# Autodesk Inventor assembly: Assembly1
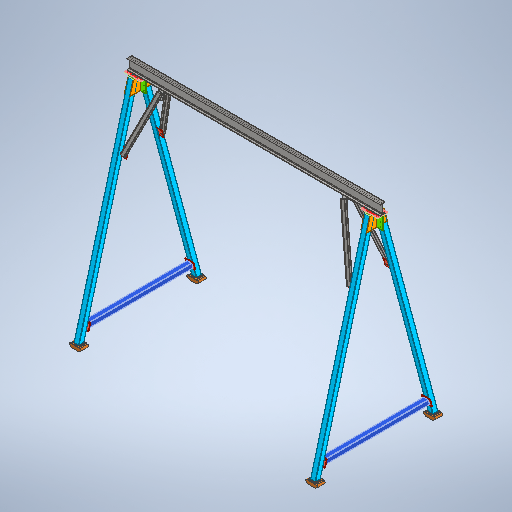
[picture p0: Inventor's stored thumbnail of the model, 512x512]
Saved by Autodesk Inventor 2025 (Build 290162010, 162A)
## iProperties
Created: 2024-06-11
Part Number: Assembly1
Document SubType Name: Assembly
Designer: admin
Author: admin
## Documents named in this file (6)
- C:\Users\pokla\Documents\Inventor\Goat 1\Assembly1.iam
- C:\Users\pokla\Documents\Inventor\Goat 1\WRS 000,000 кран козловой 6х4.ipt
- C:\Users\pokla\Documents\Inventor\Goat 1\Тельфер Таль электрическая.ipt
- C:\Users\pokla\Documents\Inventor\Goat 1\Сrane plate 1.ipt
- C:\Users\pokla\Documents\Inventor\Goat 1\Assembly2 стойка.iam
- C:\Users\pokla\Documents\Inventor\Goat 1\Двутавр 240x36 - 6000.ipt
## Components (7 placed, 7 different names)
1. WRS 000,000 кран козловой 6х4.ipt:1 — Mate:2, Mate:3, Flush:3
2. Тельфер Таль электрическая.ipt:1 — Mate:4
3. Сrane plate 1.ipt:1 — Flush:18
4. Assembly2 стойка.iam:1 [sub-assembly] — Flush:24, Flush:25, Flush:26
5. Двутавр 240x36 - 6000:1 — Mate:7, Mate:8, Flush:28
6. Assembly2 стойка:2 [sub-assembly] — Flush:27, Mate:5, Mate:6, Rigid:3
7. Сrane plate 1:2 — Rigid:3, Mate:8
## Relationships (18: Flush 9, Mate 7, WeldJoint 2)
- Mate:2: WRS 000,000 кран козловой 6х4.ipt:1
- Mate:3: WRS 000,000 кран козловой 6х4.ipt:1
- Flush:3: WRS 000,000 кран козловой 6х4.ipt:1
- Mate:4: Тельфер Таль электрическая.ipt:1
- [Flush]: Assembly2 стойка.iam:1
- Flush:18: Сrane plate 1.ipt:1
- [Flush]: Assembly2 стойка.iam:1
- [WeldJoint]: Сrane plate 1.ipt:1 ↔ Assembly2 стойка.iam:1
- Flush:24: Assembly2 стойка.iam:1
- Flush:25: Assembly2 стойка.iam:1
- Flush:26 (-2800 mm): Assembly2 стойка.iam:1
- Flush:27: Assembly2 стойка:2
- Mate:5: Assembly2 стойка:2
- Mate:6 (-2800 mm): Assembly2 стойка:2
- Rigid:3 [WeldJoint]: Assembly2 стойка:2 ↔ Сrane plate 1:2
- Mate:7: Двутавр 240x36 - 6000:1
- Mate:8: Двутавр 240x36 - 6000:1 ↔ Сrane plate 1:2
- Flush:28: Двутавр 240x36 - 6000:1
